# Autodesk Inventor assembly: Assembly
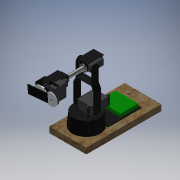
[picture p0: Inventor's stored thumbnail of the model, 180x180]
Saved by Autodesk Inventor 2017 (Build 210142000, 142)
## iProperties
Created: 2018-10-14
Part Number: Assembly
Document SubType Name: Assembly
Designer: Cameron
Author: Cameron
## Documents named in this file (19)
- C:\Users\Cameron\Desktop\Robotics\Assembly.iam
- C:\Users\Cameron\Desktop\Robotics\Base.ipt
- C:\Users\Cameron\Desktop\Robotics\Electronics Plate.ipt
- C:\Users\Cameron\Desktop\Robotics\Motherboard.ipt
- C:\Users\Cameron\Desktop\Robotics\Rotating Top.ipt
- C:\Users\Cameron\Desktop\Robotics\Shoulder Plate.ipt
- C:\Users\Cameron\Desktop\Robotics\Shoulder Servo.ipt
- C:\Users\Cameron\Desktop\Robotics\Wooden Base.ipt
- C:\Users\Cameron\Desktop\Robotics\Upper Arm.ipt
- C:\Users\Cameron\Desktop\Robotics\elbow servo plate.ipt
- C:\Users\Cameron\Desktop\Robotics\Elbow Servo.ipt
- C:\Users\Cameron\Desktop\Robotics\linkage connector.ipt
- C:\Users\Cameron\Desktop\Robotics\Middle Arm Linkage.ipt
- C:\Users\Cameron\Desktop\Robotics\Wrist U-Plate.ipt
- C:\Users\Cameron\Desktop\Robotics\Wrist Servo Plate.ipt
- C:\Users\Cameron\Desktop\Robotics\Wrist Bearing.ipt
- C:\Users\Cameron\Desktop\Robotics\Wrist Sprocket.ipt
- C:\Users\Cameron\Desktop\Robotics\Wrist Standoff.ipt
- C:\Users\Cameron\Desktop\Robotics\Hand Plate.ipt
## Components (26 placed, 18 different names)
1. Base:1 — Mate:1, Mate:2, Mate:3, Mate:5, Mate:7, Mate:8
2. Electronics Plate:1 — Mate:4, Mate:5, Mate:6, Flush:1, Flush:2
3. Motherboard:1 — Mate:6, Flush:1, Flush:2
4. Rotating Top:1 — Mate:7, Mate:8, Mate:9, Mate:10, Mate:11
5. Shoulder Plate:1 — Mate:9, Mate:10, Mate:11, Mate:12, Mate:13, Mate:14
6. Shoulder Servo:1 — Mate:12, Mate:13, Mate:14, Mate:15, Mate:16
7. Wooden Base:1 — Mate:1, Mate:2, Mate:3, Mate:4
8. Upper Arm:1 — Mate:15, Mate:16, Mate:22, Mate:23
9. elbow servo plate:1 — Mate:19, Mate:20, Mate:21, Mate:24, Mate:25, Flush:3
10. Elbow Servo:1 — Mate:19, Mate:20, Mate:21, Mate:22, Mate:23
11. linkage connector:1 — Mate:24, Mate:25, Flush:3, Mate:26, Mate:27, Flush:4
12. linkage connector:2 — Mate:28, Mate:29, Flush:4, Mate:30, Mate:31, Flush:5
13. Middle Arm Linkage:1 — Mate:26, Mate:27, Mate:28, Mate:29
14. elbow servo plate:2 — Mate:30, Mate:31, Flush:5, Mate:32, Mate:33, Mate:34
15. Elbow Servo:2 — Mate:32, Mate:33, Mate:34, Mate:35, Mate:36
16. Wrist U-Plate:1 — Mate:35, Mate:36, Mate:37, Mate:38, Flush:6
17. Wrist Servo Plate:1 — Mate:37, Mate:38, Flush:6, Mate:39, Mate:40, Mate:41, Mate:42, Mate:43, Mate:44
18. Elbow Servo:3 — Mate:39, Mate:40, Mate:41, Flush:7, Mate:57
19. Wrist Bearing:1 — Mate:55, Mate:56, Mate:58, Mate:59, Mate:60
20. Wrist Bearing:2 — Mate:42, Mate:43, Mate:44, Mate:52, Mate:53, Mate:54
21. Wrist Bearing:3 — Mate:52, Mate:53, Mate:54, Mate:55, Mate:56
22. Wrist Sprocket:1 — Mate:58, Mate:59, Mate:60, Mate:61, Mate:62, Mate:63, Mate:64
23. Wrist Sprocket:2 — Flush:7, Mate:57
24. Wrist Standoff:1 — Mate:62, Mate:63, Mate:65
25. Wrist Standoff:2 — Mate:61, Mate:64, Mate:66, Mate:67
26. Hand Plate:1 — Mate:65, Mate:66, Mate:67
## Relationships (65: Mate 58, Flush 7)
- Mate:1: Base:1 ↔ Wooden Base:1
- Mate:2 (-65 mm): Base:1 ↔ Wooden Base:1
- Mate:3 (-65 mm): Base:1 ↔ Wooden Base:1
- Mate:4: Electronics Plate:1 ↔ Wooden Base:1
- Mate:5: Base:1 ↔ Electronics Plate:1
- Mate:6: Electronics Plate:1 ↔ Motherboard:1
- Flush:1 (5 mm): Electronics Plate:1 ↔ Motherboard:1
- Flush:2 (-5 mm): Electronics Plate:1 ↔ Motherboard:1
- Mate:7: Base:1 ↔ Rotating Top:1
- Mate:8: Base:1 ↔ Rotating Top:1
- Mate:9: Rotating Top:1 ↔ Shoulder Plate:1
- Mate:10 (-20 mm): Rotating Top:1 ↔ Shoulder Plate:1
- Mate:11 (-20 mm): Rotating Top:1 ↔ Shoulder Plate:1
- Mate:12: Shoulder Plate:1 ↔ Shoulder Servo:1
- Mate:13: Shoulder Plate:1 ↔ Shoulder Servo:1
- Mate:14: Shoulder Plate:1 ↔ Shoulder Servo:1
- Mate:15: Shoulder Servo:1 ↔ Upper Arm:1
- Mate:16: Shoulder Servo:1 ↔ Upper Arm:1
- Mate:19: elbow servo plate:1 ↔ Elbow Servo:1
- Mate:20: elbow servo plate:1 ↔ Elbow Servo:1
- Mate:21: elbow servo plate:1 ↔ Elbow Servo:1
- Mate:22: Upper Arm:1 ↔ Elbow Servo:1
- Mate:23: Upper Arm:1 ↔ Elbow Servo:1
- Mate:24: elbow servo plate:1 ↔ linkage connector:1
- Mate:25: elbow servo plate:1 ↔ linkage connector:1
- Flush:3: elbow servo plate:1 ↔ linkage connector:1
- Mate:26: linkage connector:1 ↔ Middle Arm Linkage:1
- Mate:27: linkage connector:1 ↔ Middle Arm Linkage:1
- Mate:28: linkage connector:2 ↔ Middle Arm Linkage:1
- Mate:29: linkage connector:2 ↔ Middle Arm Linkage:1
- Flush:4: linkage connector:1 ↔ linkage connector:2
- Mate:30: linkage connector:2 ↔ elbow servo plate:2
- Mate:31: linkage connector:2 ↔ elbow servo plate:2
- Flush:5: linkage connector:2 ↔ elbow servo plate:2
- Mate:32: elbow servo plate:2 ↔ Elbow Servo:2
- Mate:33: elbow servo plate:2 ↔ Elbow Servo:2
- Mate:34: elbow servo plate:2 ↔ Elbow Servo:2
- Mate:35: Elbow Servo:2 ↔ Wrist U-Plate:1
- Mate:36: Elbow Servo:2 ↔ Wrist U-Plate:1
- Mate:37: Wrist U-Plate:1 ↔ Wrist Servo Plate:1
- Mate:38: Wrist U-Plate:1 ↔ Wrist Servo Plate:1
- Flush:6: Wrist U-Plate:1 ↔ Wrist Servo Plate:1
- Mate:39: Wrist Servo Plate:1 ↔ Elbow Servo:3
- Mate:40: Wrist Servo Plate:1 ↔ Elbow Servo:3
- Mate:41: Wrist Servo Plate:1 ↔ Elbow Servo:3
- Mate:42: Wrist Servo Plate:1 ↔ Wrist Bearing:2
- Mate:43: Wrist Servo Plate:1 ↔ Wrist Bearing:2
- Mate:44: Wrist Servo Plate:1 ↔ Wrist Bearing:2
- Mate:52: Wrist Bearing:2 ↔ Wrist Bearing:3
- Mate:53: Wrist Bearing:2 ↔ Wrist Bearing:3
- Mate:54: Wrist Bearing:2 ↔ Wrist Bearing:3
- Mate:55: Wrist Bearing:1 ↔ Wrist Bearing:3
- Mate:56: Wrist Bearing:1 ↔ Wrist Bearing:3
- Flush:7: Elbow Servo:3 ↔ Wrist Sprocket:2
- Mate:57: Elbow Servo:3 ↔ Wrist Sprocket:2
- Mate:58: Wrist Bearing:1 ↔ Wrist Sprocket:1
- Mate:59: Wrist Bearing:1 ↔ Wrist Sprocket:1
- Mate:60: Wrist Bearing:1 ↔ Wrist Sprocket:1
- Mate:61: Wrist Sprocket:1 ↔ Wrist Standoff:2
- Mate:62: Wrist Sprocket:1 ↔ Wrist Standoff:1
- Mate:63: Wrist Sprocket:1 ↔ Wrist Standoff:1
- Mate:64: Wrist Sprocket:1 ↔ Wrist Standoff:2
- Mate:65: Wrist Standoff:1 ↔ Hand Plate:1
- Mate:66: Wrist Standoff:2 ↔ Hand Plate:1
- Mate:67: Wrist Standoff:2 ↔ Hand Plate:1
